# Autodesk Inventor assembly: ASSEMBLY_Bias_Tee
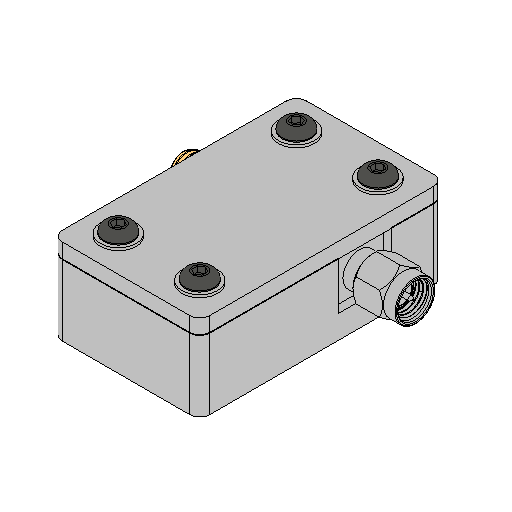
[picture p0: Inventor's stored thumbnail of the model, 512x512]
Saved by Autodesk Inventor 2026.1 (Build 301233000, 233)
## iProperties
Created: 2025-06-27
Part Number: ASSEMBLY_Bias_Tee
Document SubType Name: Assembly
Designer: User
Author: User
## Documents named in this file (7)
- C:\Users\Andrzej\OneDrive\_DRIVE_SYNCH_FILES\__ BYTECHLAB PROJECTS\RF - Mostly 3D Printed Discone Antenna\MCAD\15_DISCONE_V4_KICAD\ASSEMBLY_BIAS_TEE_REVA\ASSEMBLY_Bias_Tee.iam
- C:\Users\Andrzej\OneDrive\_DRIVE_SYNCH_FILES\__ BYTECHLAB PROJECTS\RF - Mostly 3D Printed Discone Antenna\MCAD\15_DISCONE_V4_KICAD\ASSEMBLY_BIAS_TEE_REVA\3DP_ASA_Bias_Tee_Case_Bottom.ipt
- C:\Users\Andrzej\OneDrive\_DRIVE_SYNCH_FILES\__ BYTECHLAB PROJECTS\RF - Mostly 3D Printed Discone Antenna\MCAD\15_DISCONE_V4_KICAD\__COTS_PARTS\COTS_BOSSARD_1386867_M3_Insert.ipt
- C:\Users\Andrzej\OneDrive\_DRIVE_SYNCH_FILES\__ BYTECHLAB PROJECTS\RF - Mostly 3D Printed Discone Antenna\MCAD\15_DISCONE_V4_KICAD\ASSEMBLY_BIAS_TEE_REVA\3DP_ASA_Bias_Tee_Case_Top.ipt
- C:\Users\Andrzej\OneDrive\_DRIVE_SYNCH_FILES\__ BYTECHLAB PROJECTS\RF - Mostly 3D Printed Discone Antenna\MCAD\15_DISCONE_V4_KICAD\__CONTENT_CENTER_PARTS\en-US\DIN 125-1  A\DIN 125 - A 3,2.ipt
- C:\Users\Andrzej\OneDrive\_DRIVE_SYNCH_FILES\__ BYTECHLAB PROJECTS\RF - Mostly 3D Printed Discone Antenna\MCAD\15_DISCONE_V4_KICAD\__CONTENT_CENTER_PARTS\en-US\ISO 7380-1\ISO 7380-1 - M3 x 12.ipt
- C:\Users\Andrzej\OneDrive\_DRIVE_SYNCH_FILES\__ BYTECHLAB PROJECTS\RF - Mostly 3D Printed Discone Antenna\MCAD\15_DISCONE_V4_KICAD\__KICAD_PCB_PARTS\4_BIAS_TEE_PCB\ASSEMBLY_BIAS_TEE_PCB.iam
## Components (15 placed, 6 different names)
1. 3DP_ASA_Bias_Tee_Case_Bottom:1 — Mate:1, Mate:2, Mate:3, Mate:4, Flush:1, Flush:2, Flush:3, Flush:4, Flush:5, Flush:6, Mate:5
2. COTS_BOSSARD_1386867_M3_Insert:1 — Mate:4, Flush:1, Mate:7
3. COTS_BOSSARD_1386867_M3_Insert:2 — Mate:3, Flush:2
4. COTS_BOSSARD_1386867_M3_Insert:3 — Mate:2, Flush:3
5. COTS_BOSSARD_1386867_M3_Insert:4 — Mate:1, Flush:4, Mate:6
6. 3DP_ASA_Bias_Tee_Case_Top:1 — Flush:5, Flush:6, Insert:1, Insert:2, Insert:3, Insert:4, Mate:8
7. DIN 125-1 A A 3,2:1 — Insert:1, Insert:5
8. DIN 125-1 A A 3,2:2 — Insert:2, Insert:7
9. DIN 125-1 A A 3,2:3 — Insert:3, Insert:6
10. DIN 125-1 A A 3,2:4 — Insert:4, Insert:8
11. ISO 7380-1 M3 x 12:1 — Insert:5
12. ISO 7380-1 M3 x 12:2 — Insert:6
13. ISO 7380-1 M3 x 12:3 — Insert:7
14. ISO 7380-1 M3 x 12:4 — Insert:8
15. ASSEMBLY_BIAS_TEE_PCB:1 [sub-assembly] — Mate:5, Mate:6, Mate:7, Mate:8
## Relationships (22: Mate 8, Insert 8, Flush 6)
- Mate:1: 3DP_ASA_Bias_Tee_Case_Bottom:1 ↔ COTS_BOSSARD_1386867_M3_Insert:4
- Mate:2: 3DP_ASA_Bias_Tee_Case_Bottom:1 ↔ COTS_BOSSARD_1386867_M3_Insert:3
- Mate:3: 3DP_ASA_Bias_Tee_Case_Bottom:1 ↔ COTS_BOSSARD_1386867_M3_Insert:2
- Mate:4: 3DP_ASA_Bias_Tee_Case_Bottom:1 ↔ COTS_BOSSARD_1386867_M3_Insert:1
- Flush:1: 3DP_ASA_Bias_Tee_Case_Bottom:1 ↔ COTS_BOSSARD_1386867_M3_Insert:1
- Flush:2: 3DP_ASA_Bias_Tee_Case_Bottom:1 ↔ COTS_BOSSARD_1386867_M3_Insert:2
- Flush:3: 3DP_ASA_Bias_Tee_Case_Bottom:1 ↔ COTS_BOSSARD_1386867_M3_Insert:3
- Flush:4: 3DP_ASA_Bias_Tee_Case_Bottom:1 ↔ COTS_BOSSARD_1386867_M3_Insert:4
- Flush:5: 3DP_ASA_Bias_Tee_Case_Bottom:1 ↔ 3DP_ASA_Bias_Tee_Case_Top:1
- Flush:6: 3DP_ASA_Bias_Tee_Case_Bottom:1 ↔ 3DP_ASA_Bias_Tee_Case_Top:1
- Insert:1: 3DP_ASA_Bias_Tee_Case_Top:1 ↔ DIN 125-1 A A 3,2:1
- Insert:2: 3DP_ASA_Bias_Tee_Case_Top:1 ↔ DIN 125-1 A A 3,2:2
- Insert:3: 3DP_ASA_Bias_Tee_Case_Top:1 ↔ DIN 125-1 A A 3,2:3
- Insert:4: 3DP_ASA_Bias_Tee_Case_Top:1 ↔ DIN 125-1 A A 3,2:4
- Insert:5: DIN 125-1 A A 3,2:1 ↔ ISO 7380-1 M3 x 12:1
- Insert:6: DIN 125-1 A A 3,2:3 ↔ ISO 7380-1 M3 x 12:2
- Insert:7: DIN 125-1 A A 3,2:2 ↔ ISO 7380-1 M3 x 12:3
- Insert:8: DIN 125-1 A A 3,2:4 ↔ ISO 7380-1 M3 x 12:4
- Mate:5: 3DP_ASA_Bias_Tee_Case_Bottom:1 ↔ ASSEMBLY_BIAS_TEE_PCB:1
- Mate:6: COTS_BOSSARD_1386867_M3_Insert:4 ↔ ASSEMBLY_BIAS_TEE_PCB:1
- Mate:7: COTS_BOSSARD_1386867_M3_Insert:1 ↔ ASSEMBLY_BIAS_TEE_PCB:1
- Mate:8: 3DP_ASA_Bias_Tee_Case_Top:1 ↔ ASSEMBLY_BIAS_TEE_PCB:1
